# Autodesk Inventor assembly: Keilverbindung2
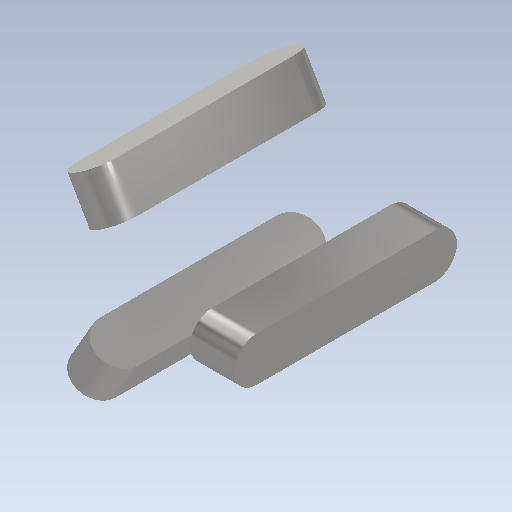
[picture p0: Inventor's stored thumbnail of the model, 512x512]
Saved by Autodesk Inventor 2021 (Build 250183000, 183)
## iProperties
ClientObjectVersion: 1
Created: 2021-01-19
Part Number: Keilverbindung2
Document SubType Name: Assembly
Designer: Jaro Machnow
Author: Jaro Machnow
## Documents named in this file (2)
- C:\Users\Jaro Machnow\Documents\Vault\Gruppen\Gruppe 2\Entwurf\Amphibienfahrzeug\Wechsel zwischen Land und Wasser\Wechselmechanik\Klappmechanismus\Keilverbindung2.iam
- C:\Users\Jaro Machnow\Documents\Inventor\Content Center Files\R2021\de-DE\DIN 6885-1 A\DIN 6885 - A 2 x 2 x 10.ipt
## Components (3 placed, 1 different names)
1. DIN 6885-1 A A 2 x 2 x 10:1
2. DIN 6885-1 A A 2 x 2 x 10:2
3. DIN 6885-1 A A 2 x 2 x 10:3
## Component patterns: (3 elements, first: DIN 6885-1 A A 2 x 2 x 10:1)
